# Autodesk Inventor assembly: structure_rear
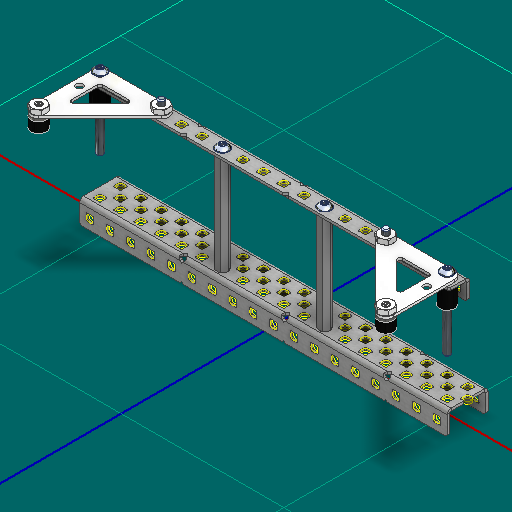
[picture p0: Inventor's stored thumbnail of the model, 512x512]
Saved by Autodesk Inventor 2025 (Build 290162000, 162)
## iProperties
Created: 2024-08-21
Part Number: structure_rear
Document SubType Name: Assembly
Designer: averey
Author: averey
## Documents named in this file (7)
- C:\Users\avere\vex_robotics_high_stakes\hardware\cad\bots\ENIGMA\chassis\drivetrain\structure\structure_rear.iam
- C:\Users\avere\vex_robotics_high_stakes\hardware\cad\VEX-CAD-Inventor\Structure\C Channel\Aluminum 1x2x1\Alu C 1x2x1x18.ipt
- C:\Users\avere\vex_robotics_high_stakes\hardware\cad\VEX-CAD-Inventor\Structure\Standoff\Standoff 2.50.ipt
- C:\Users\avere\vex_robotics_high_stakes\hardware\cad\VEX-CAD-Inventor\Structure\Standoff.ipt
- C:\Users\avere\vex_robotics_high_stakes\hardware\cad\VEX-CAD-Inventor\Structure\Hardware\Screw Shoulder Robosource\SScrew Shoulder Smooth .500 x .04.ipt
- C:\Users\avere\vex_robotics_high_stakes\hardware\cad\VEX-CAD-Inventor\Structure\Hardware\Screw Shoulder Robosource.ipt
- C:\Users\avere\vex_robotics_high_stakes\hardware\cad\bots\ENIGMA\chassis\drivetrain\structure\angle_triangle_brace.iam
## Components (8 placed, 4 different names)
1. Alu C 1x2x1x18:1 — Mate:2, Insert:9, Insert:10
2. Standoff 2.50:1 — Mate:3
3. Standoff 2.50:2 — Insert:11
4. SScrew Shoulder Smooth .500 x .04:1 — Insert:13
5. SScrew Shoulder Smooth .500 x .04:2 — Insert:12
6. SScrew Shoulder Smooth .500 x .04:3 — Insert:9
7. SScrew Shoulder Smooth .500 x .04:4 — Insert:10
8. angle_triangle_brace:1 [sub-assembly] — Insert:11, Mate:3, Insert:12, Insert:13
## Relationships (9: Insert 7, Mate 2)
- [Insert]: Alu C 1x2x1x18:1 ↔ Standoff 2.50:2
- [Insert]: Alu C 1x2x1x18:1 ↔ Standoff 2.50:1
- Mate:2: Alu C 1x2x1x18:1
- Insert:9: Alu C 1x2x1x18:1 ↔ SScrew Shoulder Smooth .500 x .04:3
- Insert:10: Alu C 1x2x1x18:1 ↔ SScrew Shoulder Smooth .500 x .04:4
- Insert:11: Standoff 2.50:2 ↔ angle_triangle_brace:1
- Mate:3: Standoff 2.50:1 ↔ angle_triangle_brace:1
- Insert:12: SScrew Shoulder Smooth .500 x .04:2 ↔ angle_triangle_brace:1
- Insert:13: SScrew Shoulder Smooth .500 x .04:1 ↔ angle_triangle_brace:1
